# Autodesk Inventor assembly: Zespół1
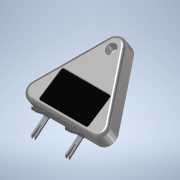
[picture p0: Inventor's stored thumbnail of the model, 180x180]
Saved by Autodesk Inventor 2020 (Build 240168000, 168)
## iProperties
Created: 2019-11-17
Part Number: Zespół1
Material: Ogólny
Document SubType Name: Assembly
Designer: macie
Author: macie
## Documents named in this file (7)
- C:\Users\hubslo\Desktop\fotobudka\fotobudka\Zespół1.iam
- D:\Pulpit\rp4\Raspberry Pi 4 Model B.ipt
- C:\Users\hubslo\Desktop\fotobudka\fotobudka\obudowa.ipt
- C:\Users\hubslo\Desktop\fotobudka\fotobudka\WIATRAK.ipt
- C:\Users\hubslo\Desktop\fotobudka\fotobudka\noga.ipt
- C:\Users\hubslo\Desktop\raspberry-pi-4-model-b-1.snapshot.3\Raspberry Pi 4 Model B.iam
- C:\Users\hubslo\Desktop\fotobudka\fotobudka\ekran.ipt
## Components (7 placed, 5 different names)
1. Raspberry Pi 4 Model B:1 — Zestawiające:1, Zestawiające:2
2. obudowa:1 — Zestawiające:1, Zestawiające:2, Zestawiające:3, Zestawiające:4, Zestawiające:6, Zestawiające:7, Zestawiające:8, Zestawiające:9, Zestawiające:10, Zestawiające:12, Zestawiające:13, Kątowe:1, Zestawiające:14, Kątowe:2, Zestawiające:15, Zestawiające:16
3. WIATRAK:1 — Zestawiające:12, Zestawiające:13, Kątowe:1
4. noga:1 — Zestawiające:3, Zestawiające:4
5. noga:2 — Zestawiające:6, Zestawiające:7
6. Raspberry Pi 4 Model B:2 [sub-assembly] — Zestawiające:8, Zestawiające:9, Zestawiające:10
7. ekran:1 — Zestawiające:14, Kątowe:2, Zestawiające:15, Zestawiające:16
## Relationships (16: Mate 14, Angle 2)
- Zestawiające:1 [Mate]: Raspberry Pi 4 Model B:1 ↔ obudowa:1
- Zestawiające:2 [Mate]: Raspberry Pi 4 Model B:1 ↔ obudowa:1
- Zestawiające:3 [Mate]: obudowa:1 ↔ noga:1
- Zestawiające:4 [Mate]: obudowa:1 ↔ noga:1
- Zestawiające:6 [Mate]: obudowa:1 ↔ noga:2
- Zestawiające:7 [Mate]: obudowa:1 ↔ noga:2
- Zestawiające:8 [Mate]: obudowa:1 ↔ Raspberry Pi 4 Model B:2
- Zestawiające:9 [Mate]: obudowa:1 ↔ Raspberry Pi 4 Model B:2
- Zestawiające:10 [Mate]: obudowa:1 ↔ Raspberry Pi 4 Model B:2
- Zestawiające:12 [Mate]: obudowa:1 ↔ WIATRAK:1
- Zestawiające:13 [Mate]: obudowa:1 ↔ WIATRAK:1
- Kątowe:1 [Angle] (0 deg): obudowa:1 ↔ WIATRAK:1
- Zestawiające:14 [Mate]: obudowa:1 ↔ ekran:1
- Kątowe:2 [Angle] (0 deg): obudowa:1 ↔ ekran:1
- Zestawiające:15 [Mate] (-2 mm): obudowa:1 ↔ ekran:1
- Zestawiające:16 [Mate] (-2 mm): obudowa:1 ↔ ekran:1
